# Autodesk Inventor assembly: rear light mount
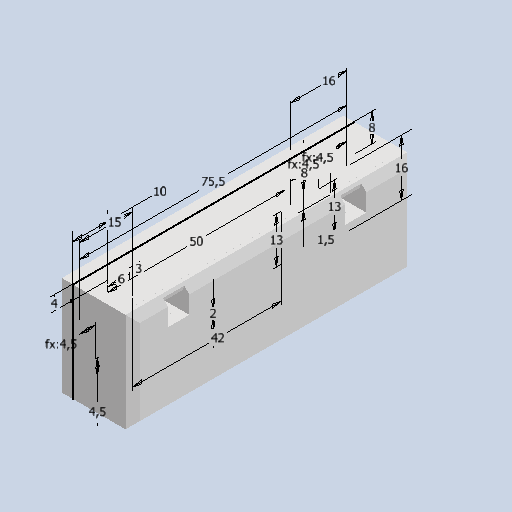
[picture p0: Inventor's stored thumbnail of the model, 512x512]
Saved by Autodesk Inventor 2022.2 (Build 262287000, 287)
## iProperties
Created: 2022-04-24
Part Number: rear light mount
Document SubType Name: Assembly
Designer: foriw
Author: foriw
## Documents named in this file (3)
- H:\inventor ting\Mekatronik beercart git\Beercart CAD\Workspaces\Workspace\rear light mount.iam
- H:\inventor ting\Mekatronik beercart git\Beercart CAD\Workspaces\Workspace\rearlightMount.ipt
- H:\inventor ting\Mekatronik beercart git\Beercart CAD\Workspaces\Workspace\rear lightcover.ipt
## Components (2 placed, 2 different names)
1. rearlightMount:1
2. rear lightcover:1
## Relationships (1: Flush 1)
- [Flush]: rearlightMount:1 ↔ rear lightcover:1
